# Autodesk Inventor assembly: 足全体
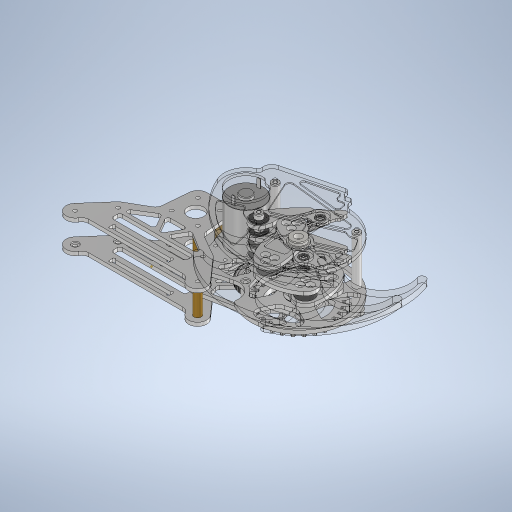
[picture p0: Inventor's stored thumbnail of the model, 512x512]
Saved by Autodesk Inventor 2023 (Build 270158000, 158)
## iProperties
Created: 2022-01-30
Part Number: 足全体
Document SubType Name: Assembly
Designer: acps
Author: acps
## Documents named in this file (4)
- C:\Users\acps\Documents\srdc\srdc_ksh\脚\足全体.iam
- C:\Users\acps\Documents\srdc\srdc_ksh\脚\足ユニット.iam
- C:\Users\acps\Documents\srdc\srdc_ksh\脚\中間ユニット内.ipt
- C:\Users\acps\Documents\srdc\srdc_ksh\スペーサ\l23.ipt
## Components (7 placed, 3 different names)
1. 足ユニット:1 [sub-assembly] — Mate:1, Insert:1, Insert:2
2. 中間ユニット内:1 — Mate:1, Insert:1, Mate:2, Mate:3, Insert:3, Insert:4, Insert:5, Insert:6
3. 中間ユニット内:2 — Mate:2, Mate:3, Insert:2
4. l23:1 — Insert:3
5. l23:2 — Insert:5
6. l23:3 — Insert:4
7. l23:4 — Insert:6
## Relationships (9: Insert 6, Mate 3)
- Mate:1: 足ユニット:1 ↔ 中間ユニット内:1
- Insert:1: 足ユニット:1 ↔ 中間ユニット内:1
- Mate:2: 中間ユニット内:1 ↔ 中間ユニット内:2
- Mate:3: 中間ユニット内:1 ↔ 中間ユニット内:2
- Insert:2: 足ユニット:1 ↔ 中間ユニット内:2
- Insert:3: 中間ユニット内:1 ↔ l23:1
- Insert:4: 中間ユニット内:1 ↔ l23:3
- Insert:5: 中間ユニット内:1 ↔ l23:2
- Insert:6: 中間ユニット内:1 ↔ l23:4
